# Autodesk Inventor assembly: assembly
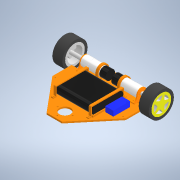
[picture p0: Inventor's stored thumbnail of the model, 180x180]
Saved by Autodesk Inventor 2020.3 (Build 243373000, 373)
## iProperties
Created: 2020-06-30
Part Number: assembly
Document SubType Name: Assembly
Designer: Devin
Author: Devin
## Documents named in this file (9)
- C:\Github\robo_car\mechanical\assembly.iam
- C:\Github\robo_car\mechanical\bp_v2.ipt
- C:\Github\robo_car\mechanical\main_motor_mount.ipt
- C:\Github\robo_car\mechanical\gearmotor.ipt
- C:\Github\robo_car\mechanical\motor_support.ipt
- C:\Github\robo_car\mechanical\anker_battery_pack.ipt
- C:\Github\robo_car\mechanical\battery_pack_clamp.ipt
- C:\Github\robo_car\mechanical\boost_converter.ipt
- C:\Github\robo_car\mechanical\mock_wheel.ipt
## Components (13 placed, 8 different names)
1. bp_v2:1 — Flush:1, Rigid:1, Flush:2, Rigid:2, Mate:3, Mate:4, Rigid:3, Rigid:4, Mate:10, Rigid:5, Mate:12, Mate:13
2. main_motor_mount:2 — Flush:1, Rigid:1, Mate:1, Cylindrical:1
3. main_motor_mount:3 — Flush:2, Rigid:2, Mate:2, Cylindrical:2
4. gearmotor:2 — Mate:1, Cylindrical:1, Rotational:1
5. gearmotor:3 — Mate:2, Cylindrical:2, Rotational:2
6. motor_support:1 — Mate:3, Rigid:4
7. motor_support:2 — Mate:4, Rigid:3
8. anker_battery_pack:1 — Mate:10, Rigid:5, Rigid:6, Rigid:7
9. battery_pack_clamp:1 — Rigid:6
10. battery_pack_clamp:2 — Mate:12, Rigid:7
11. boost_converter:1 — Mate:13
12. mock_wheel:1 — Rotational:1
13. mock_wheel:2 — Rotational:2
## Relationships (20: WeldJoint 7, Mate 7, Flush 2, CylindricalJoint 2, RevoluteJoint 2)
- Flush:1: bp_v2:1 ↔ main_motor_mount:2
- Rigid:1 [WeldJoint]: bp_v2:1 ↔ main_motor_mount:2
- Flush:2: bp_v2:1 ↔ main_motor_mount:3
- Rigid:2 [WeldJoint]: bp_v2:1 ↔ main_motor_mount:3
- Mate:1: main_motor_mount:2 ↔ gearmotor:2
- Cylindrical:1: main_motor_mount:2 ↔ gearmotor:2
- Mate:2: main_motor_mount:3 ↔ gearmotor:3
- Cylindrical:2: main_motor_mount:3 ↔ gearmotor:3
- Mate:3: bp_v2:1 ↔ motor_support:1
- Mate:4: bp_v2:1 ↔ motor_support:2
- Rigid:3 [WeldJoint]: bp_v2:1 ↔ motor_support:2
- Rigid:4 [WeldJoint]: bp_v2:1 ↔ motor_support:1
- Mate:10: bp_v2:1 ↔ anker_battery_pack:1
- Rigid:5 [WeldJoint]: bp_v2:1 ↔ anker_battery_pack:1
- Mate:12: bp_v2:1 ↔ battery_pack_clamp:2
- Rigid:6 [WeldJoint]: anker_battery_pack:1 ↔ battery_pack_clamp:1
- Rigid:7 [WeldJoint]: anker_battery_pack:1 ↔ battery_pack_clamp:2
- Mate:13: bp_v2:1 ↔ boost_converter:1
- Rotational:1 [RevoluteJoint]: gearmotor:2 ↔ mock_wheel:1
- Rotational:2 [RevoluteJoint]: gearmotor:3 ↔ mock_wheel:2
